# Autodesk Inventor assembly: PrzekladniaPrawa
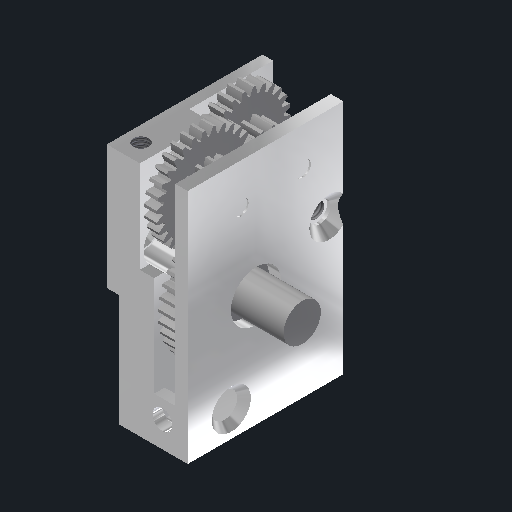
[picture p0: Inventor's stored thumbnail of the model, 512x512]
Saved by Autodesk Inventor 2023 (Build 270158000, 158)
## iProperties
Created: 2022-03-19
Part Number: PrzekladniaPrawa
Material: Ogólny
Document SubType Name: Assembly
Designer: Michał
Mass: 32.6535 g
Surface Area: 77.3749 cm^2
Volume: 7.75156 cm^3
Density: 4.21251 g/cm^3
Author: Michał
## Documents named in this file (7)
- D:\Projekty\RoboIlo\Ser\3D\3D\PrzekladniaPrawa.iam
- D:\Projekty\RoboIlo\Ser\3D\3D\MocowaniePrawejPrzekladni.ipt
- D:\Projekty\RoboIlo\Ser\3D\3D\PrzekladniaLewa\Design Accelerator\Przekładnie walcowe2.iam
- D:\Projekty\RoboIlo\Ser\3D\3D\PrzekladniaLewa\Design Accelerator\Przekładnie walcowe3.iam
- D:\Projekty\RoboIlo\Ser\3D\3D\PrzekladniaLewa\Design Accelerator\Przekładnie walcowe4.iam
- D:\Projekty\RoboIlo\Ser\3D\3D\Oś.ipt
- D:\Projekty\RoboIlo\Ser\3D\3D\OslonaPrawejPrzekladni.ipt
## Components (7 placed, 4 different names)
1. MocowaniePrawejPrzekladni:1 — Zestawiający:1, Zestawiający:2, Zestawiający:3, Zestawiający:4, Wstaw:3, Wstaw:4, Równoległy:1, Zestawiający:5
2. Przekładnie walcowe:1 [sub-assembly] — Wstaw:1, Zestawiający:1, Zestawiający:5
3. Przekładnie walcowe:2 [sub-assembly] — Wstaw:1, Wstaw:2, Zestawiający:2
4. Przekładnie walcowe:3 [sub-assembly] — Wstaw:2, Zestawiający:3, Zestawiający:4
5. Oś:1 — Wstaw:4
6. Oś:2 — Wstaw:3
7. OslonaPrawejPrzekladni:1 — Równoległy:1
## Relationships (10: Mate 5, Insert 4, Flush 1)
- Wstaw:1 [Insert]: Przekładnie walcowe:1 ↔ Przekładnie walcowe:2
- Wstaw:2 [Insert]: Przekładnie walcowe:2 ↔ Przekładnie walcowe:3
- Zestawiający:1 [Mate]: MocowaniePrawejPrzekladni:1 ↔ Przekładnie walcowe:1
- Zestawiający:2 [Mate]: MocowaniePrawejPrzekladni:1 ↔ Przekładnie walcowe:2
- Zestawiający:3 [Mate]: MocowaniePrawejPrzekladni:1 ↔ Przekładnie walcowe:3
- Zestawiający:4 [Mate]: MocowaniePrawejPrzekladni:1 ↔ Przekładnie walcowe:3
- Wstaw:3 [Insert]: MocowaniePrawejPrzekladni:1 ↔ Oś:2
- Wstaw:4 [Insert]: MocowaniePrawejPrzekladni:1 ↔ Oś:1
- Równoległy:1 [Flush]: MocowaniePrawejPrzekladni:1 ↔ OslonaPrawejPrzekladni:1
- Zestawiający:5 [Mate] (0.1 mm): MocowaniePrawejPrzekladni:1 ↔ Przekładnie walcowe:1
